# Autodesk Inventor assembly: Traction Wheel Assembly 1764
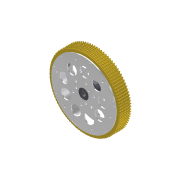
[picture p0: Inventor's stored thumbnail of the model, 180x180]
Saved by Autodesk Inventor 2011 (Build 150239000, 239)
## iProperties
Created: 2009-01-18
Part Number: Traction Wheel Assembly 1764
Document SubType Name: Assembly
Designer: pmulligan
Mass: 313.226 g
Surface Area: 2212.12 cm^2
Volume: 313.226 cm^3
Density: 1 g/cm^3
Author: pmulligan
## Documents named in this file (6)
- R:\2010-2011\CMO\Web Site\CADalog\Wheels\Large Traction Wheel 1764\Large Traction Wheel Assembly 1764.iam
- R:\2010-2011\CMO\Web Site\CADalog\Wheels\Large Traction Wheel 1764\Large Traction Tread 1764.ipt
- R:\2010-2011\CMO\Web Site\CADalog\Wheels\Large Traction Wheel 1764\Traction Wheel Brace 1764.ipt
- R:\2010-2011\CMO\Web Site\CADalog\Wheels\Large Traction Wheel 1764\Traction Mount 1764.ipt
- R:\2010-2011\CMO\Web Site\CADalog\Wheels\Large Traction Wheel 1764\Traction Wheel Side Plate 1764.ipt
- R:\2010-2011\CMO\Web Site\CADalog\Wheels\Wheel Bearing 1764\Wheel Bearing 1764.iam
## Components (12 placed, 5 different names)
1. Traction Wheel Brace 1764:1 — Mate:47, Mate:48
2. Traction Wheel Brace 1764:2 — Mate:54, Mate:55
3. Traction Wheel Brace 1764:3 — Mate:57, Mate:58
4. Traction Wheel Brace 1764:4 — Mate:60, Mate:61
5. Traction Wheel Brace 1764:5 — Mate:62, Mate:63
6. Traction Wheel Brace 1764:6 — Mate:51, Mate:52
7. Traction Mount 1764:1 — Mate:44, Mate:45, Mate:46, Mate:66, Mate:67, Mate:68, Mate:69
8. Traction Wheel Side Plate 1764:1 — Mate:44, Mate:45, Mate:46, Mate:47, Mate:48, Mate:51, Mate:52, Mate:54, Mate:55, Mate:57, Mate:58, Mate:60, Mate:61, Mate:62, Mate:63, Mate:70, Flush:2, Mate:72
9. Traction Wheel Side Plate 1764:2 — Mate:66, Mate:67, Mate:68, Mate:71, Flush:1
10. Large Traction Tread 1764:1 — Mate:69, Mate:70
11. Wheel Bearing 1764:1 [sub-assembly] — Flush:2, Mate:72
12. Wheel Bearing 1764:2 [sub-assembly] — Mate:71, Flush:1
## Relationships (24: Mate 22, Flush 2)
- Mate:44: Traction Mount 1764:1 ↔ Traction Wheel Side Plate 1764:1
- Mate:45: Traction Mount 1764:1 ↔ Traction Wheel Side Plate 1764:1
- Mate:46: Traction Mount 1764:1 ↔ Traction Wheel Side Plate 1764:1
- Mate:47: Traction Wheel Brace 1764:1 ↔ Traction Wheel Side Plate 1764:1
- Mate:48: Traction Wheel Brace 1764:1 ↔ Traction Wheel Side Plate 1764:1
- Mate:51: Traction Wheel Brace 1764:6 ↔ Traction Wheel Side Plate 1764:1
- Mate:52: Traction Wheel Brace 1764:6 ↔ Traction Wheel Side Plate 1764:1
- Mate:54: Traction Wheel Brace 1764:2 ↔ Traction Wheel Side Plate 1764:1
- Mate:55: Traction Wheel Brace 1764:2 ↔ Traction Wheel Side Plate 1764:1
- Mate:57: Traction Wheel Brace 1764:3 ↔ Traction Wheel Side Plate 1764:1
- Mate:58: Traction Wheel Brace 1764:3 ↔ Traction Wheel Side Plate 1764:1
- Mate:60: Traction Wheel Brace 1764:4 ↔ Traction Wheel Side Plate 1764:1
- Mate:61: Traction Wheel Brace 1764:4 ↔ Traction Wheel Side Plate 1764:1
- Mate:62: Traction Wheel Brace 1764:5 ↔ Traction Wheel Side Plate 1764:1
- Mate:63: Traction Wheel Brace 1764:5 ↔ Traction Wheel Side Plate 1764:1
- Mate:66: Traction Mount 1764:1 ↔ Traction Wheel Side Plate 1764:2
- Mate:67: Traction Mount 1764:1 ↔ Traction Wheel Side Plate 1764:2
- Mate:68: Traction Mount 1764:1 ↔ Traction Wheel Side Plate 1764:2
- Mate:69: Traction Mount 1764:1 ↔ Large Traction Tread 1764:1
- Mate:70: Traction Wheel Side Plate 1764:1 ↔ Large Traction Tread 1764:1
- Mate:71: Traction Wheel Side Plate 1764:2 ↔ Wheel Bearing 1764:2
- Flush:1: Traction Wheel Side Plate 1764:2 ↔ Wheel Bearing 1764:2
- Flush:2: Traction Wheel Side Plate 1764:1 ↔ Wheel Bearing 1764:1
- Mate:72: Traction Wheel Side Plate 1764:1 ↔ Wheel Bearing 1764:1
